# Autodesk Inventor assembly: gear
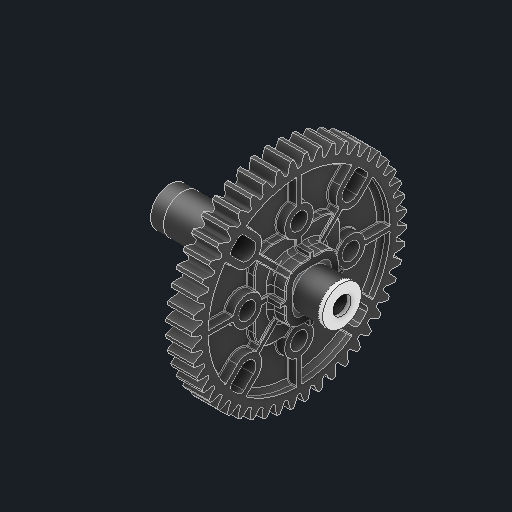
[picture p0: Inventor's stored thumbnail of the model, 512x512]
Saved by Autodesk Inventor 2025 (Build 290162000, 162)
## iProperties
Created: 2024-10-03
Part Number: gear
Document SubType Name: Assembly
Designer: Averey Ku
Author: Averey Ku
## Documents named in this file (9)
- D:\vex_robotics_high_stakes\hardware\cad\bots\high_stakes_v2\chassis\drivebay\gear.iam
- D:\vex_robotics_high_stakes\hardware\cad\robpros_cad_lib\Modified Parts\modified_parts\Half Cut HS 48T Gear, No Insert.ipt
- D:\vex_robotics_high_stakes\hardware\cad\robpros_cad_lib\Motion\Spacers\Spacer Nylon .375 OD\NSpacer .375 OD x .250.ipt
- D:\vex_robotics_high_stakes\hardware\cad\robpros_cad_lib\Motion\Spacers\Spacer Nylon .375 OD.ipt
- D:\vex_robotics_high_stakes\hardware\cad\robpros_cad_lib\Motion\Spacers\Washer Teflon\TWasher .375 OD x .04000.ipt
- D:\vex_robotics_high_stakes\hardware\cad\robpros_cad_lib\Motion\Spacers\Washer Teflon.ipt
- D:\vex_robotics_high_stakes\hardware\cad\robpros_cad_lib\Motion\Spacers\Spacer Nylon .375 OD\NSpacer .375 OD x .500.ipt
- D:\vex_robotics_high_stakes\hardware\cad\robpros_cad_lib\Motion\Shaft LS\Shaft Collar ipts\Shaft Collar Set Screw.ipt
- D:\vex_robotics_high_stakes\hardware\cad\robpros_cad_lib\Motion\Spacers\Spacer Nylon .375 OD\NSpacer .375 OD x .125.ipt
## Components (6 placed, 6 different names)
1. Half Cut HS 48T Gear, No Insert:1 — Insert:2, Insert:3
2. NSpacer .375 OD x .250:1 — Insert:1, Insert:2
3. TWasher .375 OD x .04000:1 — Insert:1
4. NSpacer .375 OD x .500:3 — Insert:4, Insert:5
5. Shaft Collar Set Screw:1 — Insert:3, Insert:4
6. NSpacer .375 OD x .125:4 — Insert:5
## Relationships (5: Insert 5)
- Insert:1: NSpacer .375 OD x .250:1 ↔ TWasher .375 OD x .04000:1
- Insert:2: Half Cut HS 48T Gear, No Insert:1 ↔ NSpacer .375 OD x .250:1
- Insert:3: Half Cut HS 48T Gear, No Insert:1 ↔ Shaft Collar Set Screw:1
- Insert:4: NSpacer .375 OD x .500:3 ↔ Shaft Collar Set Screw:1
- Insert:5: NSpacer .375 OD x .500:3 ↔ NSpacer .375 OD x .125:4
